# Autodesk Inventor assembly: MARCO CORREDERA 1400X1200 MM
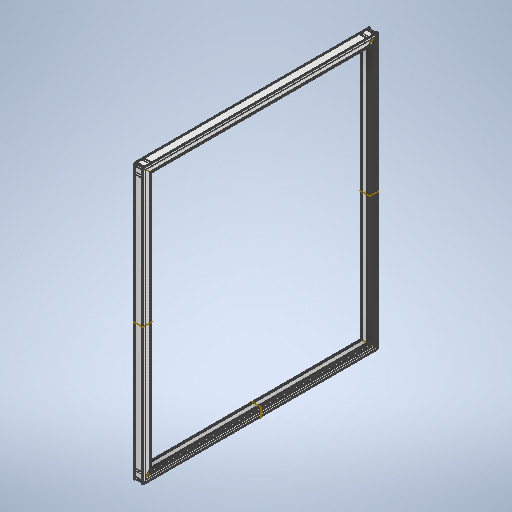
[picture p0: Inventor's stored thumbnail of the model, 512x512]
Saved by Autodesk Inventor 2025 (Build 290162000, 162)
## iProperties
Created: 2026-02-13
Part Number: MARCO CORREDERA 1400X1200 MM
Document SubType Name: Assembly
Designer: Frank
Author: Frank
## Documents named in this file (9)
- D:\Inventor\Proyectos\MARQUTERIA DE ALUMINIO\MARCO DE CORREDERA\MARCO CORREDERA 1400X1200 MM.iam
- D:\Inventor\Proyectos\MARQUTERIA DE ALUMINIO\MARCO DE CORREDERA\SP40-09 MARCO CORREDERA 1400 MM.ipt
- D:\Inventor\Proyectos\MARQUTERIA DE ALUMINIO\MARCO DE CORREDERA\SP40-09 MARCO CORREDERA 1200 MM.ipt
- D:\Inventor\Proyectos\MARQUTERIA DE ALUMINIO\GENERAL\ESCUADRA UNIÓN 45 FINA.ipt
- D:\Inventor\Proyectos\MARQUTERIA DE ALUMINIO\MARCO DE CORREDERA\SP40-09 MARCO CORREDERA 1200 MM_MIR.ipt
- D:\Inventor\Proyectos\MARQUTERIA DE ALUMINIO\MARCO DE CORREDERA\ESCUADRA UNIÓN 45 FINA_MIR.ipt
- D:\Inventor\Proyectos\MARQUTERIA DE ALUMINIO\MARCO DE CORREDERA\SP40-09 MARCO CORREDERA 1400 MM_MIR.ipt
- D:\Inventor\Proyectos\MARQUTERIA DE ALUMINIO\MARCO DE CORREDERA\ESCUADRA UNIÓN 45 FINA_MIR1.ipt
- D:\Inventor\Proyectos\MARQUTERIA DE ALUMINIO\MARCO DE CORREDERA\ESCUADRA UNIÓN 45 FINA_MIR_MIR.ipt
## Components (8 placed, 8 different names)
1. SP40-09 MARCO CORREDERA 1400 MM:1 — Coincidencia:1, Coincidencia:2, Coincidencia:4
2. SP40-09 MARCO CORREDERA 1200 MM:1 — Coincidencia:3, Coincidencia:4
3. ESCUADRA UNIÓN 45 FINA:1 — Coincidencia:1, Coincidencia:2, Coincidencia:3
4. SP40-09 MARCO CORREDERA 1200 MM_MIR:1 — Coincidencia:5
5. ESCUADRA UNIÓN 45 FINA_MIR:1 — Coincidencia:5
6. SP40-09 MARCO CORREDERA 1400 MM_MIR:1 — Coincidencia:6, Coincidencia:7
7. ESCUADRA UNIÓN 45 FINA_MIR1:1 — Coincidencia:6, Coincidencia:7
8. ESCUADRA UNIÓN 45 FINA_MIR_MIR:1
## Relationships (7: Mate 7)
- Coincidencia:1 [Mate]: SP40-09 MARCO CORREDERA 1400 MM:1 ↔ ESCUADRA UNIÓN 45 FINA:1
- Coincidencia:2 [Mate] (1 mm): SP40-09 MARCO CORREDERA 1400 MM:1 ↔ ESCUADRA UNIÓN 45 FINA:1
- Coincidencia:3 [Mate]: SP40-09 MARCO CORREDERA 1200 MM:1 ↔ ESCUADRA UNIÓN 45 FINA:1
- Coincidencia:4 [Mate]: SP40-09 MARCO CORREDERA 1400 MM:1 ↔ SP40-09 MARCO CORREDERA 1200 MM:1
- Coincidencia:5 [Mate]: SP40-09 MARCO CORREDERA 1200 MM_MIR:1 ↔ ESCUADRA UNIÓN 45 FINA_MIR:1
- Coincidencia:6 [Mate] (1 mm): SP40-09 MARCO CORREDERA 1400 MM_MIR:1 ↔ ESCUADRA UNIÓN 45 FINA_MIR1:1
- Coincidencia:7 [Mate]: SP40-09 MARCO CORREDERA 1400 MM_MIR:1 ↔ ESCUADRA UNIÓN 45 FINA_MIR1:1
